# Autodesk Inventor assembly: Assembly1
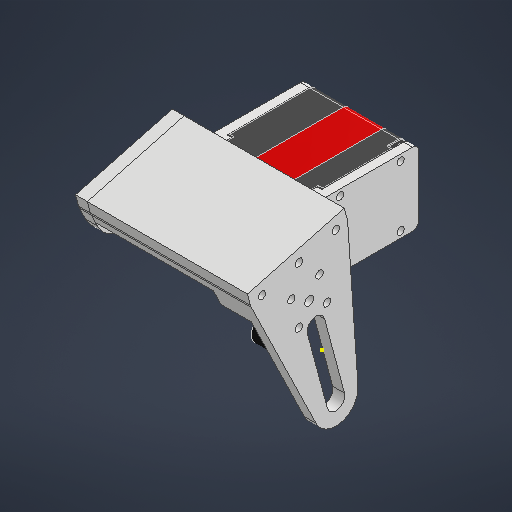
[picture p0: Inventor's stored thumbnail of the model, 512x512]
Saved by Autodesk Inventor 2026 (Build 300175000, 175)
## iProperties
Created: 2025-12-05
Part Number: Assembly1
Document SubType Name: Assembly
Designer: numai
Author: numai
## Documents named in this file (7)
- C:\Users\numai\Documents\workspace\inventor\feetech_slider_3dprint\Assembly1.iam
- C:\Users\numai\Documents\workspace\inventor\feetech_slider_3dprint\HLS3950M.ipt
- C:\Users\numai\Documents\workspace\inventor\feetech_slider_3dprint\ARRMA_1_7_25t_servo_arm.ipt
- C:\Users\numai\Documents\workspace\inventor\feetech_slider_3dprint\servo_side_plate1.ipt
- C:\Users\numai\Documents\workspace\inventor\feetech_slider_3dprint\servo_side_plate2.ipt
- C:\Users\numai\Documents\workspace\inventor\feetech_slider_3dprint\guideline.ipt
- C:\Users\numai\Documents\workspace\inventor\feetech_slider_3dprint\guideline_mir.ipt
## Components (6 placed, 6 different names)
1. HLS3950M:1 — メイト:1, メイト:2, フラッシュ:1, フラッシュ:2, フラッシュ:3
2. ARRMA_1_7_25t_servo_arm:1 — メイト:1, メイト:2, メイト:4, メイト:9
3. servo_side_plate1:1 — フラッシュ:1, フラッシュ:2, メイト:3
4. servo_side_plate2:1 — フラッシュ:3
5. guideline:1 — メイト:3, メイト:4, メイト:6, メイト:7, メイト:8, メイト:9
6. guideline_mir:1 — メイト:6, メイト:7, メイト:8
## Relationships (11: Mate 8, Flush 3)
- メイト:1 [Mate]: HLS3950M:1 ↔ ARRMA_1_7_25t_servo_arm:1
- メイト:2 [Mate] (0.4 mm): HLS3950M:1 ↔ ARRMA_1_7_25t_servo_arm:1
- フラッシュ:1 [Flush]: HLS3950M:1 ↔ servo_side_plate1:1
- フラッシュ:2 [Flush]: HLS3950M:1 ↔ servo_side_plate1:1
- フラッシュ:3 [Flush]: HLS3950M:1 ↔ servo_side_plate2:1
- メイト:3 [Mate]: servo_side_plate1:1 ↔ guideline:1
- メイト:4 [Mate] (3 mm): ARRMA_1_7_25t_servo_arm:1 ↔ guideline:1
- メイト:6 [Mate]: guideline:1 ↔ guideline_mir:1
- メイト:7 [Mate]: guideline:1 ↔ guideline_mir:1
- メイト:8 [Mate]: guideline:1 ↔ guideline_mir:1
- メイト:9 [Mate]: ARRMA_1_7_25t_servo_arm:1 ↔ guideline:1
